# Autodesk Inventor assembly: HBLFSD5-SEC
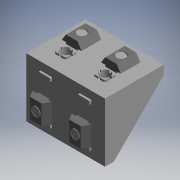
[picture p0: Inventor's stored thumbnail of the model, 180x180]
Saved by Autodesk Inventor 2017.3 (Build 213256000, 256)
## iProperties
Category: PARTsolutions
Company: MISUMI
Part Number: HBLFSD5-SEC
Catalog Web Link: www.cadenas.de
Description: HBLFSD5-Brackets HFS5 Reversal Brackets with Tab 2 Slots
Vendor: MISUMI
Document SubType Name: Assembly
Designer: partserver
Manufacturer: MISUMI
Mass: 13.8726 g
Surface Area: 111.863 cm^2
Volume: 13.8726 cm^3
Density: 1 g/cm^3
Title: HBLFSD5-SEC
Author: Cadenas PARTsolutions
Comments: Brackets HFS5 Reversal Brackets with Tab 2 Slots
PSOL_IDENT_0: {$CADENAS_DATA\23d-libs\misumi\metric\38_al_extrusions_blackets\5\hblfsd5_asmtab.prj},178 {VTYP=3D},
PSOL_IDENT_1: {STYP=ASSTAB},{NB=HBLFSD5-SEC},{LINA=HBLFSD5-SEC},{NN=HBLFSD5},{DATE=09.09.2019 15:28:10},{GEOMDATE=
PSOL_IDENT_2: 08.09.2009},{VERSION=},{LINEID=270},{WBVAR=ALT1,ALT2},{WBNUMERIC=}  {NB=HBLFSD5-SEC},{LINA=HBLFSD5-S
PSOL_IDENT_3: EC},{KT=7},{PN=HBLFSD5-SEC},{TP=HBLFSD5},{NOH=2},{NOHV=2},{MAT=ADC12},{ST=-},{TYPE=HBLFSD5},{FEAT=Re
PSOL_IDENT_4: versal Bracket with Tab},{ALT1=},{ALT2=-SEC},{MASS=25},{AB=HCBST5-12},{NOB=4},{AN=HNTT5-5},{NON=4},{
PSOL_IDENT_5: AL=1470},{W=40},{H=30},{DP=30},{T=4.5},{HDIS=0},{DPOS=12},{HH1=18},{HV1=0},{DIA=5.2},{ALT1OPT='','w/
PSOL_IDENT_6: o C (Mounting Holes for Cover)','-C','with C (Mounting Holes for Cover)'},{ALT2OPT= '' , 'w/o Set of
PSOL_IDENT_7: Applicable Bolt and Nut' , '-SET' , 'with SET (Set of Applicable Bolt and Nut)' , '-SST' , 'with SS
PSOL_IDENT_8: T (Stainless Steel Set of Applicable Bolt and Nut)' , '-SEU' , 'with SEU (Pre-Assembly Fitting Sprin
PSOL_IDENT_9: g Nuts Set of Applicable Bolt and Nut)' , '-SSU' , 'with SSU (Pre-Assembly Fitting Spring Nuts Stain
PSOL_IDENT_10: less Set of Applicable Bolt and Nut)'  , '-SEP' , 'with SEP (Post-Assembly Fitting Spring Nuts Set o
PSOL_IDENT_11: f Applicable Bolt and Nut)' , '-SSP' , 'with SSP (Post-Assembly Fitting Spring Nuts Stainless Set of
PSOL_IDENT_12: Applicable Bolt and Nut)' , '-SEC' , 'with SEC (Washer Assembled Set of Applicable Bolt and Nut)' }
PSOL_IDENT_13: ,{R=1},{R1=0.3},{APOSV=0},{VER=3},{PR=7},{TT=1.0},{T1=0},{TIP=HBLFSN5},{PPATH=hblfsl5_asmtpl.prj},{A
PSOL_IDENT_14: BT=HCBST5-},{ABL=12}
NB: HBLFSD5-SEC
NN: HBLFSD5
NT: Brackets HFS5 Reversal Brackets with Tab 2 Slots
NBSYN: $PN.
LINA: HBLFSD5-SEC
CATALOG: Misumi
PN: HBLFSD5-SEC
MAT: ADC12
ST: -
FEAT: Reversal Bracket with Tab
ALT1: w/o C (Mounting Holes for Cover)
ALT2: with SEC (Washer Assembled Set of Applicable Bolt and Nut)
MASS: 25
AB: HCBST5-12
NOB: 4
AN: HNTT5-5
NON: 4
AL: 1470
SUPPLIER: MISUMI
ARTICLENO: HBLFSD5-SEC
BOMINFO: HBLFSD5-SEC
CREATOR: CADENAS GmbH
## Documents named in this file (6)
- e:\temp\worker_17\temp\exporttempdir_7780_10_Ao9X5\format_0\HBLFSD5-SEC.iam
- e:\temp\worker_17\temp\exporttempdir_7780_10_Ao9X5\format_0\HBLFSD5-SECh5.ipt
- e:\temp\worker_17\temp\exporttempdir_7780_10_Ao9X5\format_0\HCBST5-12_Screw.ipt
- e:\temp\worker_17\temp\exporttempdir_7780_10_Ao9X5\format_0\HCBST5_w1.ipt
- e:\temp\worker_17\temp\exporttempdir_7780_10_Ao9X5\format_0\SPWF5.ipt
- e:\temp\worker_17\temp\exporttempdir_7780_10_Ao9X5\format_0\HNTT5-5_1.ipt
## Components (17 placed, 5 different names)
1. HBLFSD5-SECh5:1 — to_bolt_row_10_11_1_Z@1 <-> screw_to_body_Z@2, to_bolt_row_10_11_2_Z@1 <-> screw_to_body_Z@3, to_bolt_row_10_11_1_Z@1 <-> spring_washer_to_bolt_Z@4, to_bolt_row_10_11_2_Z@1 <-> spring_washer_to_bolt_Z@5, to_bolt_row_10_11_1_Z@1 <-> plain_washer_to_bolt_Z@6, to_bolt_row_10_11_2_Z@1 <-> plain_washer_to_bolt_Z@7, to_bolt_row_10_11_1_Z@1 <-> to_frames_Z@8, to_bolt_row_10_11_2_Z@1 <-> to_frames_Z@9, bolt_10_11_base_1_Z@1 <-> screw_to_body_Z@10, bolt_10_11_base_2_Z@1 <-> screw_to_body_Z@11, bolt_10_11_base_1_Z@1 <-> spring_washer_to_bolt_Z@12, bolt_10_11_base_2_Z@1 <-> spring_washer_to_bolt_Z@13, bolt_10_11_base_1_Z@1 <-> plain_washer_to_bolt_Z@14, bolt_10_11_base_2_Z@1 <-> plain_washer_to_bolt_Z@15, bolt_10_11_base_1_Z@1 <-> to_frames_Z@16, bolt_10_11_base_2_Z@1 <-> to_frames_Z@17
2. HCBST5-12_Screw:1 — to_bolt_row_10_11_1_Z@1 <-> screw_to_body_Z@2
3. HCBST5-12_Screw:2 — to_bolt_row_10_11_2_Z@1 <-> screw_to_body_Z@3
4. HCBST5_w1:1 — to_bolt_row_10_11_1_Z@1 <-> spring_washer_to_bolt_Z@4
5. HCBST5_w1:2 — to_bolt_row_10_11_2_Z@1 <-> spring_washer_to_bolt_Z@5
6. SPWF5:1 — to_bolt_row_10_11_1_Z@1 <-> plain_washer_to_bolt_Z@6
7. SPWF5:2 — to_bolt_row_10_11_2_Z@1 <-> plain_washer_to_bolt_Z@7
8. HNTT5-5_1:1 — to_bolt_row_10_11_1_Z@1 <-> to_frames_Z@8
9. HNTT5-5_1:2 — to_bolt_row_10_11_2_Z@1 <-> to_frames_Z@9
10. HCBST5-12_Screw:3 — bolt_10_11_base_1_Z@1 <-> screw_to_body_Z@10
11. HCBST5-12_Screw:4 — bolt_10_11_base_2_Z@1 <-> screw_to_body_Z@11
12. HCBST5_w1:3 — bolt_10_11_base_1_Z@1 <-> spring_washer_to_bolt_Z@12
13. HCBST5_w1:4 — bolt_10_11_base_2_Z@1 <-> spring_washer_to_bolt_Z@13
14. SPWF5:3 — bolt_10_11_base_1_Z@1 <-> plain_washer_to_bolt_Z@14
15. SPWF5:4 — bolt_10_11_base_2_Z@1 <-> plain_washer_to_bolt_Z@15
16. HNTT5-5_1:3 — bolt_10_11_base_1_Z@1 <-> to_frames_Z@16
17. HNTT5-5_1:4 — bolt_10_11_base_2_Z@1 <-> to_frames_Z@17
## Relationships (16: Mate 16)
- to_bolt_row_10_11_1_Z@1 <-> screw_to_body_Z@2 [Mate]: HBLFSD5-SECh5:1 ↔ HCBST5-12_Screw:1
- to_bolt_row_10_11_2_Z@1 <-> screw_to_body_Z@3 [Mate]: HBLFSD5-SECh5:1 ↔ HCBST5-12_Screw:2
- to_bolt_row_10_11_1_Z@1 <-> spring_washer_to_bolt_Z@4 [Mate]: HBLFSD5-SECh5:1 ↔ HCBST5_w1:1
- to_bolt_row_10_11_2_Z@1 <-> spring_washer_to_bolt_Z@5 [Mate]: HBLFSD5-SECh5:1 ↔ HCBST5_w1:2
- to_bolt_row_10_11_1_Z@1 <-> plain_washer_to_bolt_Z@6 [Mate]: HBLFSD5-SECh5:1 ↔ SPWF5:1
- to_bolt_row_10_11_2_Z@1 <-> plain_washer_to_bolt_Z@7 [Mate]: HBLFSD5-SECh5:1 ↔ SPWF5:2
- to_bolt_row_10_11_1_Z@1 <-> to_frames_Z@8 [Mate]: HBLFSD5-SECh5:1 ↔ HNTT5-5_1:1
- to_bolt_row_10_11_2_Z@1 <-> to_frames_Z@9 [Mate]: HBLFSD5-SECh5:1 ↔ HNTT5-5_1:2
- bolt_10_11_base_1_Z@1 <-> screw_to_body_Z@10 [Mate]: HBLFSD5-SECh5:1 ↔ HCBST5-12_Screw:3
- bolt_10_11_base_2_Z@1 <-> screw_to_body_Z@11 [Mate]: HBLFSD5-SECh5:1 ↔ HCBST5-12_Screw:4
- bolt_10_11_base_1_Z@1 <-> spring_washer_to_bolt_Z@12 [Mate]: HBLFSD5-SECh5:1 ↔ HCBST5_w1:3
- bolt_10_11_base_2_Z@1 <-> spring_washer_to_bolt_Z@13 [Mate]: HBLFSD5-SECh5:1 ↔ HCBST5_w1:4
- bolt_10_11_base_1_Z@1 <-> plain_washer_to_bolt_Z@14 [Mate]: HBLFSD5-SECh5:1 ↔ SPWF5:3
- bolt_10_11_base_2_Z@1 <-> plain_washer_to_bolt_Z@15 [Mate]: HBLFSD5-SECh5:1 ↔ SPWF5:4
- bolt_10_11_base_1_Z@1 <-> to_frames_Z@16 [Mate]: HBLFSD5-SECh5:1 ↔ HNTT5-5_1:3
- bolt_10_11_base_2_Z@1 <-> to_frames_Z@17 [Mate]: HBLFSD5-SECh5:1 ↔ HNTT5-5_1:4
